# Autodesk Inventor assembly: Konarm_3_przegub_v2
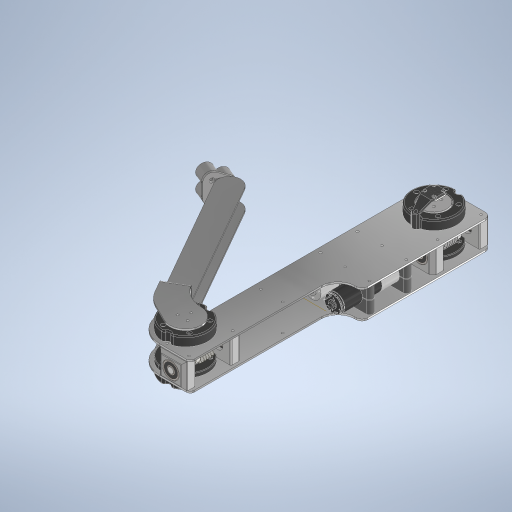
[picture p0: Inventor's stored thumbnail of the model, 512x512]
Saved by Autodesk Inventor 2023 (Build 270158000, 158)
## iProperties
Created: 2023-01-27
Part Number: Konarm_3_przegub_v2
Document SubType Name: Assembly
Designer: Kamil
Mass: 929.155 g
Surface Area: 4430.92 cm^2
Volume: 901.223 cm^3
Density: 1.03099 g/cm^3
Author: Kamil
## Documents named in this file (23)
- C:\Users\Kamil\Desktop\KONARM\konarm 3 przegub\Konarm_3_przegub_v2.iam
- C:\Users\Kamil\Desktop\KONARM\konarm 3 przegub\blacha.ipt
- C:\Users\Kamil\Desktop\KONARM\konarm 3 przegub\koszyczek.ipt
- C:\Users\Kamil\Desktop\KONARM\konarm 3 przegub\kolnierz wewnetrzny.ipt
- C:\Users\Kamil\Desktop\KONARM\konarm 3 przegub\Złożenie2.STEP.ipt
- C:\Users\Kamil\Desktop\KONARM\konarm 3 przegub\Faulhaber 3272G012C R.ipt
- C:\Users\Kamil\Desktop\KONARM\konarm 3 przegub\os_napedowa.ipt
- C:\Users\Kamil\Desktop\KONARM\konarm 3 przegub\Os.ipt
- C:\Users\Kamil\Desktop\KONARM\konarm 3 przegub\Os_lewa.ipt
- C:\Users\Kamil\Desktop\KONARM\konarm 3 przegub\kółko.ipt
- C:\Users\Kamil\Desktop\KONARM\konarm 3 przegub\ball bearing(6006).ipt
- C:\Users\Kamil\Desktop\KONARM\konarm 3 przegub\blacha_MIR.ipt
- C:\Users\Kamil\Desktop\KONARM\konarm 3 przegub\blacha_2.ipt
- C:\Users\Kamil\Desktop\KONARM\konarm 3 przegub\Ariadna-Electromagnet_mount_v2.ipt
- C:\Users\Kamil\Desktop\KONARM\konarm 3 przegub\Złożenie2.STEP_MIR.ipt
- C:\Users\Kamil\Desktop\KONARM\konarm 3 przegub\blacha_2_MIR1.ipt
- C:\Users\Kamil\Desktop\KONARM\konarm 3 przegub\Uchwyt_na_lozysko_2.ipt
- C:\Users\Kamil\Desktop\KONARM\konarm 3 przegub\Uchwyt_na_lozysko_poli.ipt
- C:\Users\Kamil\Downloads\3200_2rs.ipt
- C:\Users\Kamil\Desktop\KONARM\Uchwyt_na_enkoder.ipt
- C:\Users\Kamil\Desktop\KONARM\AS5600 v1.ipt
- C:\Users\Kamil\Desktop\KONARM\wał_2.ipt
- C:\Users\Kamil\Desktop\KONARM\uchwyt_na_silniki_v2.ipt
## Components (48 placed, 22 different names)
1. blacha:2 — Zestawiające:64, Równoległe:1, Równoległe:2, Zestawiające:65, Zestawiające:66, Zestawiające:67, Zestawiające:68, Zestawiające:69, Zestawiające:70, Zestawiające:71, Zestawiające:72, Zestawiające:73, Zestawiające:74, Zestawiające:75, Zestawiające:76, Zestawiające:77, Zestawiające:78, Zestawiające:79, Zestawiające:80, Zestawiające:81, Zestawiające:82, Zestawiające:87, Zestawiające:102, Zestawiające:104, Równoległe:4, Zestawiające:113, Zestawiające:116, Zestawiające:117
2. koszyczek:1 — Zestawiające:36, Zestawiające:37, Zestawiające:38, Zestawiające:39, Zestawiające:60
3. koszyczek:2 — Zestawiające:77, Zestawiające:78, Zestawiające:79
4. kolnierz wewnetrzny:1 — Zestawiające:61, Zestawiające:62, Zestawiające:63
5. kolnierz wewnetrzny:2 — Zestawiające:67, Zestawiające:68, Zestawiające:69
6. Złożenie2.STEP:1
7. Faulhaber 3272G012C R:1
8. os_napedowa:1 — Zestawiające:14, Zestawiające:22
9. Os:1 — Zestawiające:43, Zestawiające:46, Zestawiające:47, Zestawiające:85
10. Os_lewa:1 — Zestawiające:83, Zestawiające:84, Zestawiające:85, Zestawiające:88, Zestawiające:91, Zestawiające:112
11. ball bearing(6006):1 — Zestawiające:73, Zestawiające:74, Zestawiające:92, Zestawiające:93, Zestawiające:95, Zestawiające:96
12. ball bearing(6006):2 — Zestawiające:27, Zestawiające:28, Zestawiające:43, Zestawiające:46, Zestawiające:48, Zestawiające:49
13. blacha_MIR:1 — Zestawiające:9, Zestawiające:11, Zestawiające:12, Zestawiające:13, Zestawiające:15, Zestawiające:16, Zestawiające:17, Zestawiające:19, Zestawiające:20, Zestawiające:21, Zestawiające:23, Zestawiające:24, Zestawiające:25, Zestawiające:27, Zestawiające:28, Zestawiające:29, Zestawiające:30, Zestawiające:35, Zestawiające:36, Zestawiające:37, Zestawiające:38, Zestawiające:39, Zestawiające:41, Zestawiające:42, Zestawiające:58, Zestawiające:59, Zestawiające:61, Równoległe:1, Równoległe:2, Zestawiające:101, Zestawiające:103, Zestawiające:114, Zestawiające:115, Zestawiające:118, Zestawiające:119, Zestawiające:120, Zestawiające:121
14. blacha_2:1 — Zestawiające:89, Zestawiające:90, Zestawiające:91, Zestawiające:98, Zestawiające:99
15. Ariadna-Electromagnet_mount_v2:1 — Zestawiające:98, Zestawiające:99
16. Złożenie2.STEP_MIR:2 — Zestawiające:9, Zestawiające:10
17. Faulhaber 3272G012C R:2 — Zestawiające:10, Zestawiające:18, Zestawiające:26, Równoległe:3
18. koszyczek:3 — Zestawiające:70, Zestawiające:71, Zestawiające:72
19. ball bearing(6006):3 — Zestawiające:75, Zestawiające:76, Zestawiające:83, Zestawiające:84, Zestawiające:86
20. kółko:3 — Zestawiające:47, Zestawiające:50, Zestawiające:51, Zestawiające:56, Zestawiające:100
21. Os_lewa:2 — Zestawiające:92, Zestawiające:93, Zestawiające:94, Zestawiające:97
22. Os:2 — Zestawiające:44, Zestawiające:45, Zestawiające:54, Zestawiające:94
23. kolnierz wewnetrzny:3 — Zestawiające:80, Zestawiające:81, Zestawiające:82
24. koszyczek:4 — Zestawiające:35, Zestawiające:40, Zestawiające:41, Zestawiające:42, Zestawiające:62, Zestawiające:63
25. kolnierz wewnetrzny:4 — Zestawiające:58, Zestawiające:59, Zestawiające:60
26. ball bearing(6006):4 — Zestawiające:29, Zestawiające:30, Zestawiające:40, Zestawiające:44, Zestawiające:45, Zestawiające:52, Zestawiające:53
27. kółko:4 — Zestawiające:52, Zestawiające:53, Zestawiające:54, Zestawiające:111
28. kółko:5 — Zestawiające:86, Zestawiające:87, Zestawiające:88, Zestawiające:89, Zestawiające:90
29. kółko:6 — Zestawiające:48, Zestawiające:49, Zestawiające:50, Zestawiające:51, Zestawiające:55, Zestawiające:57
30. blacha_2_MIR1:1 — Zestawiające:55, Zestawiające:56, Zestawiające:57, Zestawiające:100
31. Uchwyt_na_lozysko_2:1 — Zestawiające:3, Zestawiające:4, Zestawiające:15, Zestawiające:16, Zestawiające:17, Zestawiające:64, Zestawiające:66
32. Uchwyt_na_lozysko_poli:1 — Zestawiające:5, Zestawiające:6, Zestawiające:23, Zestawiające:24, Zestawiające:25
33. 3200_2rs:1 — Zestawiające:3, Zestawiające:4, Zestawiające:18
34. 3200_2rs:2 — Zestawiające:1, Zestawiające:2, Zestawiające:14
35. 3200_2rs:3 — Zestawiające:5, Zestawiające:6, Zestawiające:26
36. 3200_2rs:4 — Zestawiające:7, Zestawiające:8
37. Uchwyt_na_lozysko_2:2 — Zestawiające:1, Zestawiające:2, Zestawiające:11, Zestawiające:12, Zestawiające:13
38. Uchwyt_na_lozysko_poli:2 — Zestawiające:7, Zestawiające:8, Zestawiające:19, Zestawiające:20, Zestawiające:21, Zestawiające:22, Zestawiające:65
39. kółko:7 — Zestawiające:95, Zestawiające:96, Zestawiające:97
40. Uchwyt_na_enkoder:1 — Zestawiające:102, Zestawiające:104, Zestawiające:105, Zestawiające:106, Zestawiające:107
41. Uchwyt_na_enkoder:2 — Zestawiające:101, Zestawiające:103, Zestawiające:108, Zestawiające:109, Zestawiające:110
42. AS5600 v1:1 — Zestawiające:105, Zestawiające:106, Zestawiające:107, Zestawiające:112
43. AS5600 v1:2 — Zestawiające:108, Zestawiające:109, Zestawiające:110, Zestawiające:111
44. wał_2:1 — Równoległe:3
45. uchwyt_na_silniki_v2:1 — Równoległe:4
46. uchwyt_na_silniki_v2:2 — Zestawiające:115, Zestawiające:118, Zestawiające:121
47. uchwyt_na_silniki_v2:3 — Zestawiające:113, Zestawiające:116, Zestawiające:117
48. uchwyt_na_silniki_v2:4 — Zestawiające:114, Zestawiające:119, Zestawiające:120
## Relationships (121: Mate 117, Flush 4)
- Zestawiające:1 [Mate]: 3200_2rs:2 ↔ Uchwyt_na_lozysko_2:2
- Zestawiające:2 [Mate]: 3200_2rs:2 ↔ Uchwyt_na_lozysko_2:2
- Zestawiające:3 [Mate]: Uchwyt_na_lozysko_2:1 ↔ 3200_2rs:1
- Zestawiające:4 [Mate]: Uchwyt_na_lozysko_2:1 ↔ 3200_2rs:1
- Zestawiające:5 [Mate]: Uchwyt_na_lozysko_poli:1 ↔ 3200_2rs:3
- Zestawiające:6 [Mate]: Uchwyt_na_lozysko_poli:1 ↔ 3200_2rs:3
- Zestawiające:7 [Mate]: 3200_2rs:4 ↔ Uchwyt_na_lozysko_poli:2
- Zestawiające:8 [Mate]: 3200_2rs:4 ↔ Uchwyt_na_lozysko_poli:2
- Zestawiające:9 [Mate]: blacha_MIR:1 ↔ Złożenie2.STEP_MIR:2
- Zestawiające:10 [Mate]: Złożenie2.STEP_MIR:2 ↔ Faulhaber 3272G012C R:2
- Zestawiające:11 [Mate]: blacha_MIR:1 ↔ Uchwyt_na_lozysko_2:2
- Zestawiające:12 [Mate]: blacha_MIR:1 ↔ Uchwyt_na_lozysko_2:2
- Zestawiające:13 [Mate]: blacha_MIR:1 ↔ Uchwyt_na_lozysko_2:2
- Zestawiające:14 [Mate]: os_napedowa:1 ↔ 3200_2rs:2
- Zestawiające:15 [Mate]: blacha_MIR:1 ↔ Uchwyt_na_lozysko_2:1
- Zestawiające:16 [Mate]: blacha_MIR:1 ↔ Uchwyt_na_lozysko_2:1
- Zestawiające:17 [Mate]: blacha_MIR:1 ↔ Uchwyt_na_lozysko_2:1
- Zestawiające:18 [Mate]: Faulhaber 3272G012C R:2 ↔ 3200_2rs:1
- Zestawiające:19 [Mate]: blacha_MIR:1 ↔ Uchwyt_na_lozysko_poli:2
- Zestawiające:20 [Mate]: blacha_MIR:1 ↔ Uchwyt_na_lozysko_poli:2
- Zestawiające:21 [Mate]: blacha_MIR:1 ↔ Uchwyt_na_lozysko_poli:2
- Zestawiające:22 [Mate]: os_napedowa:1 ↔ Uchwyt_na_lozysko_poli:2
- Zestawiające:23 [Mate]: blacha_MIR:1 ↔ Uchwyt_na_lozysko_poli:1
- Zestawiające:24 [Mate]: blacha_MIR:1 ↔ Uchwyt_na_lozysko_poli:1
- Zestawiające:25 [Mate]: blacha_MIR:1 ↔ Uchwyt_na_lozysko_poli:1
- Zestawiające:26 [Mate]: Faulhaber 3272G012C R:2 ↔ 3200_2rs:3
- Zestawiające:27 [Mate]: ball bearing(6006):2 ↔ blacha_MIR:1
- Zestawiające:28 [Mate]: ball bearing(6006):2 ↔ blacha_MIR:1
- Zestawiające:29 [Mate]: blacha_MIR:1 ↔ ball bearing(6006):4
- Zestawiające:30 [Mate]: blacha_MIR:1 ↔ ball bearing(6006):4
- Zestawiające:35 [Mate]: blacha_MIR:1 ↔ koszyczek:4
- Zestawiające:36 [Mate]: koszyczek:1 ↔ blacha_MIR:1
- Zestawiające:37 [Mate]: koszyczek:1 ↔ blacha_MIR:1
- Zestawiające:38 [Mate]: koszyczek:1 ↔ blacha_MIR:1
- Zestawiające:39 [Mate]: koszyczek:1 ↔ blacha_MIR:1
- Zestawiające:40 [Mate]: koszyczek:4 ↔ ball bearing(6006):4
- Zestawiające:41 [Mate]: blacha_MIR:1 ↔ koszyczek:4
- Zestawiające:42 [Mate]: blacha_MIR:1 ↔ koszyczek:4
- Zestawiające:43 [Mate]: Os:1 ↔ ball bearing(6006):2
- Zestawiające:44 [Mate]: Os:2 ↔ ball bearing(6006):4
- Zestawiające:45 [Mate]: Os:2 ↔ ball bearing(6006):4
- Zestawiające:46 [Mate]: Os:1 ↔ ball bearing(6006):2
- Zestawiające:47 [Mate]: Os:1 ↔ kółko:3
- Zestawiające:48 [Mate]: ball bearing(6006):2 ↔ kółko:6
- Zestawiające:49 [Mate]: ball bearing(6006):2 ↔ kółko:6
- Zestawiające:50 [Mate]: kółko:3 ↔ kółko:6
- Zestawiające:51 [Mate]: kółko:3 ↔ kółko:6
- Zestawiające:52 [Mate]: ball bearing(6006):4 ↔ kółko:4
- Zestawiające:53 [Mate]: ball bearing(6006):4 ↔ kółko:4
- Zestawiające:54 [Mate]: Os:2 ↔ kółko:4
- Zestawiające:55 [Mate]: kółko:6 ↔ blacha_2_MIR1:1
- Zestawiające:56 [Mate]: kółko:3 ↔ blacha_2_MIR1:1
- Zestawiające:57 [Mate]: kółko:6 ↔ blacha_2_MIR1:1
- Zestawiające:58 [Mate]: blacha_MIR:1 ↔ kolnierz wewnetrzny:4
- Zestawiające:59 [Mate]: blacha_MIR:1 ↔ kolnierz wewnetrzny:4
- Zestawiające:60 [Mate]: koszyczek:1 ↔ kolnierz wewnetrzny:4
- Zestawiające:61 [Mate]: kolnierz wewnetrzny:1 ↔ blacha_MIR:1
- Zestawiające:62 [Mate]: kolnierz wewnetrzny:1 ↔ koszyczek:4
- Zestawiające:63 [Mate]: kolnierz wewnetrzny:1 ↔ koszyczek:4
- Zestawiające:64 [Mate]: blacha:2 ↔ Uchwyt_na_lozysko_2:1
- Równoległe:1 [Flush]: blacha:2 ↔ blacha_MIR:1
- Równoległe:2 [Flush]: blacha:2 ↔ blacha_MIR:1
- Zestawiające:65 [Mate]: blacha:2 ↔ Uchwyt_na_lozysko_poli:2
- Zestawiające:66 [Mate]: blacha:2 ↔ Uchwyt_na_lozysko_2:1
- Zestawiające:67 [Mate]: blacha:2 ↔ kolnierz wewnetrzny:2
- Zestawiające:68 [Mate]: blacha:2 ↔ kolnierz wewnetrzny:2
- Zestawiające:69 [Mate]: blacha:2 ↔ kolnierz wewnetrzny:2
- Zestawiające:70 [Mate]: blacha:2 ↔ koszyczek:3
- Zestawiające:71 [Mate]: blacha:2 ↔ koszyczek:3
- Zestawiające:72 [Mate]: blacha:2 ↔ koszyczek:3
- Zestawiające:73 [Mate]: blacha:2 ↔ ball bearing(6006):1
- Zestawiające:74 [Mate]: blacha:2 ↔ ball bearing(6006):1
- Zestawiające:75 [Mate]: blacha:2 ↔ ball bearing(6006):3
- Zestawiające:76 [Mate]: blacha:2 ↔ ball bearing(6006):3
- Zestawiające:77 [Mate]: blacha:2 ↔ koszyczek:2
- Zestawiające:78 [Mate]: blacha:2 ↔ koszyczek:2
- Zestawiające:79 [Mate]: blacha:2 ↔ koszyczek:2
- Zestawiające:80 [Mate]: blacha:2 ↔ kolnierz wewnetrzny:3
- Zestawiające:81 [Mate]: blacha:2 ↔ kolnierz wewnetrzny:3
- Zestawiające:82 [Mate]: blacha:2 ↔ kolnierz wewnetrzny:3
- Zestawiające:83 [Mate]: Os_lewa:1 ↔ ball bearing(6006):3
- Zestawiające:84 [Mate]: Os_lewa:1 ↔ ball bearing(6006):3
- Zestawiające:85 [Mate]: Os:1 ↔ Os_lewa:1
- Zestawiające:86 [Mate]: ball bearing(6006):3 ↔ kółko:5
- Zestawiające:87 [Mate]: blacha:2 ↔ kółko:5
- Zestawiające:88 [Mate]: Os_lewa:1 ↔ kółko:5
- Zestawiające:89 [Mate]: blacha_2:1 ↔ kółko:5
- Zestawiające:90 [Mate]: blacha_2:1 ↔ kółko:5
- Zestawiające:91 [Mate]: Os_lewa:1 ↔ blacha_2:1
- Zestawiające:92 [Mate]: ball bearing(6006):1 ↔ Os_lewa:2
- Zestawiające:93 [Mate]: ball bearing(6006):1 ↔ Os_lewa:2
- Zestawiające:94 [Mate]: Os_lewa:2 ↔ Os:2
- Zestawiające:95 [Mate]: ball bearing(6006):1 ↔ kółko:7
- Zestawiające:96 [Mate]: ball bearing(6006):1 ↔ kółko:7
- Zestawiające:97 [Mate]: Os_lewa:2 ↔ kółko:7
- Zestawiające:98 [Mate]: blacha_2:1 ↔ Ariadna-Electromagnet_mount_v2:1
- Zestawiające:99 [Mate]: blacha_2:1 ↔ Ariadna-Electromagnet_mount_v2:1
- Zestawiające:100 [Mate]: kółko:3 ↔ blacha_2_MIR1:1
- Zestawiające:101 [Mate]: blacha_MIR:1 ↔ Uchwyt_na_enkoder:2
- Zestawiające:102 [Mate]: blacha:2 ↔ Uchwyt_na_enkoder:1
- Zestawiające:103 [Mate]: blacha_MIR:1 ↔ Uchwyt_na_enkoder:2
- Zestawiające:104 [Mate]: blacha:2 ↔ Uchwyt_na_enkoder:1
- Zestawiające:105 [Mate]: Uchwyt_na_enkoder:1 ↔ AS5600 v1:1
- Zestawiające:106 [Mate]: Uchwyt_na_enkoder:1 ↔ AS5600 v1:1
- Zestawiające:107 [Mate]: Uchwyt_na_enkoder:1 ↔ AS5600 v1:1
- Zestawiające:108 [Mate]: Uchwyt_na_enkoder:2 ↔ AS5600 v1:2
- Zestawiające:109 [Mate]: Uchwyt_na_enkoder:2 ↔ AS5600 v1:2
- Zestawiające:110 [Mate]: Uchwyt_na_enkoder:2 ↔ AS5600 v1:2
- Zestawiające:111 [Mate]: kółko:4 ↔ AS5600 v1:2
- Zestawiające:112 [Mate]: Os_lewa:1 ↔ AS5600 v1:1
- Równoległe:3 [Flush]: Faulhaber 3272G012C R:2 ↔ wał_2:1
- Równoległe:4 [Flush]: blacha:2 ↔ uchwyt_na_silniki_v2:1
- Zestawiające:113 [Mate]: blacha:2 ↔ uchwyt_na_silniki_v2:3
- Zestawiające:114 [Mate]: blacha_MIR:1 ↔ uchwyt_na_silniki_v2:4
- Zestawiające:115 [Mate]: blacha_MIR:1 ↔ uchwyt_na_silniki_v2:2
- Zestawiające:116 [Mate]: blacha:2 ↔ uchwyt_na_silniki_v2:3
- Zestawiające:117 [Mate]: blacha:2 ↔ uchwyt_na_silniki_v2:3
- Zestawiające:118 [Mate]: blacha_MIR:1 ↔ uchwyt_na_silniki_v2:2
- Zestawiające:119 [Mate]: blacha_MIR:1 ↔ uchwyt_na_silniki_v2:4
- Zestawiające:120 [Mate]: blacha_MIR:1 ↔ uchwyt_na_silniki_v2:4
- Zestawiające:121 [Mate]: blacha_MIR:1 ↔ uchwyt_na_silniki_v2:2
